# Autodesk Inventor assembly: MechSwitch_Assem_V2
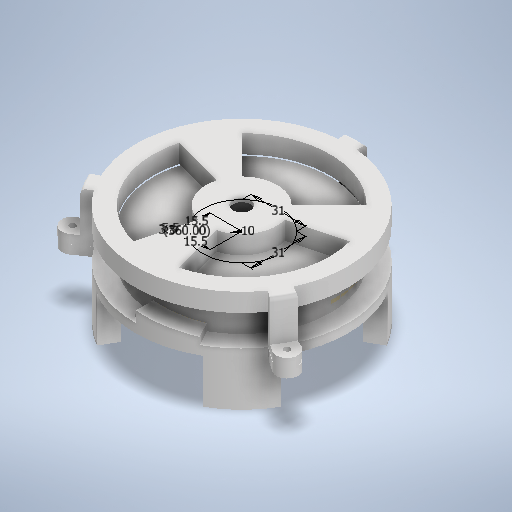
[picture p0: Inventor's stored thumbnail of the model, 512x512]
Saved by Autodesk Inventor 2025.1 (Build 291241000, 241)
## iProperties
Created: 2026-04-13
Part Number: MechSwitch_Assem_V2
Document SubType Name: Assembly
Designer: ryand
Author: ryand
## Documents named in this file (5)
- C:\Users\ryand\OneDrive\Documents\Inventor\TNG\Rotational_TENG\MechSwitch\MechSwitch_Assem_V2.iam
- C:\Users\ryand\OneDrive\Documents\Inventor\TNG\Rotational_TENG\MechSwitch\MechSwitch_DielecTopV2.ipt
- C:\Users\ryand\OneDrive\Documents\Inventor\TNG\Rotational_TENG\MechSwitch\MechSwitch_MotorBaseipt.ipt
- C:\Users\ryand\OneDrive\Documents\Inventor\TNG\Rotational_TENG\MechSwitch\Bearing-Insert.ipt
- C:\Users\ryand\OneDrive\Documents\Inventor\TNG\Rotational_TENG\MechSwitch\PCB_insert.ipt
## Components (4 placed, 4 different names)
1. MechSwitch_DielecTopV2:1 — Mate:1, Mate:2, Mate:3
2. MechSwitch_MotorBaseipt:1 — Mate:1, Mate:2, Mate:4
3. Bearing-Insert:1 — Mate:3
4. PCB_insert:1 — Mate:4
## Relationships (4: Mate 4)
- Mate:1 (0.1 mm): MechSwitch_DielecTopV2:1 ↔ MechSwitch_MotorBaseipt:1
- Mate:2 (0.1 mm): MechSwitch_DielecTopV2:1 ↔ MechSwitch_MotorBaseipt:1
- Mate:3: MechSwitch_DielecTopV2:1 ↔ Bearing-Insert:1
- Mate:4: MechSwitch_MotorBaseipt:1 ↔ PCB_insert:1
